# Autodesk Inventor assembly: ASTRAIOSV_2Assembly
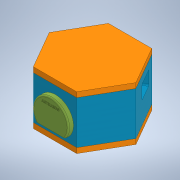
[picture p0: Inventor's stored thumbnail of the model, 180x180]
Saved by Autodesk Inventor 2020 (Build 240168000, 168)
## iProperties
Created: 2020-03-11
Part Number: ASTRAIOSV_2Assembly
Document SubType Name: Assembly
Designer: WANG
Author: WANG
## Documents named in this file (9)
- C:\Users\ianwa\Documents\GitHub\ASTRAIOS\workspace\ASTRAIOSV_2Assembly.iam
- C:\Users\ianwa\Documents\GitHub\ASTRAIOS\workspace\SatelliteBottomFace_v2.ipt
- C:\Users\ianwa\Documents\GitHub\ASTRAIOS\workspace\SatelliteSideWallPlateSensor_v2.ipt
- C:\Users\ianwa\Documents\GitHub\ASTRAIOS\workspace\SatelliteSideWallFilled_v2.ipt
- C:\Users\ianwa\Documents\GitHub\ASTRAIOS\workspace\SatelliteSideWallCamera_v2.ipt
- C:\Users\ianwa\Documents\GitHub\ASTRAIOS\workspace\SatelliteSideWallSensor_v2.ipt
- C:\Users\ianwa\Documents\GitHub\ASTRAIOS\workspace\SatelliteLexanPlate_v2.ipt
- C:\Users\ianwa\Documents\GitHub\ASTRAIOS\workspace\SatelliteTopFace_v2.ipt
- C:\Users\ianwa\Documents\GitHub\ASTRAIOS\workspace\SensorCap_v2.ipt
## Components (10 placed, 8 different names)
1. SatelliteBottomFace_v2:1 — Mate:1, Flush:1, Mate:2, Flush:2, Mate:3, Flush:3, Mate:4, Flush:4, Mate:5, Mate:6, Mate:7, Mate:8, Mate:9, Mate:10, Mate:11, Flush:5, Mate:12, Mate:13, Mate:14, Flush:6, Mate:15, Mate:16, Mate:17, Mate:18
2. SatelliteSideWallPlateSensor_v2:1 — Mate:1, Flush:1, Mate:5, Mate:7, Mate:23, Mate:24
3. SatelliteSideWallFilled_v2:1 — Mate:3, Flush:3, Mate:8, Mate:9
4. SatelliteSideWallFilled_v2:2 — Mate:2, Flush:2, Mate:6, Mate:17, Mate:18, Mate:25
5. SatelliteSideWallCamera_v2:1 — Mate:4, Flush:4, Mate:10, Mate:13
6. SatelliteSideWallFilled_v2:3 — Mate:11, Flush:5, Mate:12, Mate:15
7. SatelliteSideWallSensor_v2:1 — Mate:14, Flush:6, Mate:16, Mate:19, Flush:7, Mate:20, Mate:21
8. SatelliteLexanPlate_v2:1 — Mate:19, Flush:7, Mate:20, Mate:21
9. SatelliteTopFace_v2:1 — Mate:24, Mate:25
10. SensorCap_v2:1 — Mate:23
## Relationships (31: Mate 24, Flush 7)
- Mate:1: SatelliteBottomFace_v2:1 ↔ SatelliteSideWallPlateSensor_v2:1
- Flush:1: SatelliteBottomFace_v2:1 ↔ SatelliteSideWallPlateSensor_v2:1
- Mate:2: SatelliteBottomFace_v2:1 ↔ SatelliteSideWallFilled_v2:2
- Flush:2: SatelliteBottomFace_v2:1 ↔ SatelliteSideWallFilled_v2:2
- Mate:3: SatelliteBottomFace_v2:1 ↔ SatelliteSideWallFilled_v2:1
- Flush:3: SatelliteBottomFace_v2:1 ↔ SatelliteSideWallFilled_v2:1
- Mate:4: SatelliteBottomFace_v2:1 ↔ SatelliteSideWallCamera_v2:1
- Flush:4: SatelliteBottomFace_v2:1 ↔ SatelliteSideWallCamera_v2:1
- Mate:5: SatelliteBottomFace_v2:1 ↔ SatelliteSideWallPlateSensor_v2:1
- Mate:6: SatelliteBottomFace_v2:1 ↔ SatelliteSideWallFilled_v2:2
- Mate:7: SatelliteBottomFace_v2:1 ↔ SatelliteSideWallPlateSensor_v2:1
- Mate:8: SatelliteBottomFace_v2:1 ↔ SatelliteSideWallFilled_v2:1
- Mate:9: SatelliteBottomFace_v2:1 ↔ SatelliteSideWallFilled_v2:1
- Mate:10: SatelliteBottomFace_v2:1 ↔ SatelliteSideWallCamera_v2:1
- Mate:11: SatelliteBottomFace_v2:1 ↔ SatelliteSideWallFilled_v2:3
- Flush:5: SatelliteBottomFace_v2:1 ↔ SatelliteSideWallFilled_v2:3
- Mate:12: SatelliteBottomFace_v2:1 ↔ SatelliteSideWallFilled_v2:3
- Mate:13: SatelliteBottomFace_v2:1 ↔ SatelliteSideWallCamera_v2:1
- Mate:14: SatelliteBottomFace_v2:1 ↔ SatelliteSideWallSensor_v2:1
- Flush:6: SatelliteBottomFace_v2:1 ↔ SatelliteSideWallSensor_v2:1
- Mate:15: SatelliteBottomFace_v2:1 ↔ SatelliteSideWallFilled_v2:3
- Mate:16: SatelliteBottomFace_v2:1 ↔ SatelliteSideWallSensor_v2:1
- Mate:17: SatelliteBottomFace_v2:1 ↔ SatelliteSideWallFilled_v2:2
- Mate:18: SatelliteBottomFace_v2:1 ↔ SatelliteSideWallFilled_v2:2
- Mate:19: SatelliteSideWallSensor_v2:1 ↔ SatelliteLexanPlate_v2:1
- Flush:7: SatelliteSideWallSensor_v2:1 ↔ SatelliteLexanPlate_v2:1
- Mate:20: SatelliteSideWallSensor_v2:1 ↔ SatelliteLexanPlate_v2:1
- Mate:21: SatelliteSideWallSensor_v2:1 ↔ SatelliteLexanPlate_v2:1
- Mate:23: SatelliteSideWallPlateSensor_v2:1 ↔ SensorCap_v2:1
- Mate:24: SatelliteSideWallPlateSensor_v2:1 ↔ SatelliteTopFace_v2:1
- Mate:25: SatelliteSideWallFilled_v2:2 ↔ SatelliteTopFace_v2:1
